# Autodesk Inventor assembly: ASSEMBLY_Main_XY_Axis
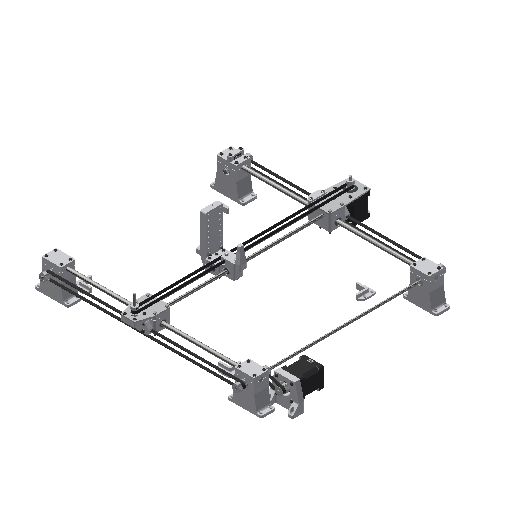
[picture p0: Inventor's stored thumbnail of the model, 512x512]
Saved by Autodesk Inventor 2025 (Build 290162010, 162A)
## iProperties
Created: 2018-06-17
Part Number: ASSEMBLY_Main_XY_Axis
Document SubType Name: Assembly
Designer: Andrzej
Author: Andrzej
## Documents named in this file (41)
- D:\_ANDRZEJ_LACZEWSKI\_OTHER\MLTDIS - SMD parts sorting machine experimental 2 axis platform\MCAD\1_REV1\ASSEMBLY_XY_AXIS_REVA\ASSEMBLY_Main_XY_Axis.iam
- D:\_ANDRZEJ_LACZEWSKI\_OTHER\MLTDIS - SMD parts sorting machine experimental 2 axis platform\MCAD\1_REV1\ASSEMBLY_XY_AXIS_REVA\CUT_STEEL_5x425mm_Linear_rod.ipt
- D:\_ANDRZEJ_LACZEWSKI\_OTHER\MLTDIS - SMD parts sorting machine experimental 2 axis platform\MCAD\1_REV1\ASSEMBLY_XY_AXIS_REVA\CUT_STEEL_6x395mm_Linear_rod.ipt
- D:\_ANDRZEJ_LACZEWSKI\_OTHER\MLTDIS - SMD parts sorting machine experimental 2 axis platform\MCAD\1_REV1\ASSEMBLY_XY_AXIS_REVA\ASSEMBLY_X_end.iam
- D:\_ANDRZEJ_LACZEWSKI\_OTHER\MLTDIS - SMD parts sorting machine experimental 2 axis platform\MCAD\1_REV1\ASSEMBLY_XY_AXIS_REVA\ASSEMBLY_X_axis_carriage.iam
- D:\_ANDRZEJ_LACZEWSKI\_OTHER\MLTDIS - SMD parts sorting machine experimental 2 axis platform\MCAD\1_REV1\ASSEMBLY_XY_AXIS_REVA\ASSEMBLY_Y_axis_motor.iam
- D:\_ANDRZEJ_LACZEWSKI\_OTHER\MLTDIS - SMD parts sorting machine experimental 2 axis platform\MCAD\1_REV1\__COTS_PARTS\COTS_GENERIC_GT2_16T_Pulley.ipt
- D:\_ANDRZEJ_LACZEWSKI\_OTHER\MLTDIS - SMD parts sorting machine experimental 2 axis platform\MCAD\1_REV1\ASSEMBLY_XY_AXIS_REVA\LC_ALU_3mm_X_axis_belt_idler_mount_plate.ipt
- D:\_ANDRZEJ_LACZEWSKI\_OTHER\MLTDIS - SMD parts sorting machine experimental 2 axis platform\MCAD\1_REV1\__COTS_PARTS\COTS_AST_695HZZ_Bearing.ipt
- D:\_ANDRZEJ_LACZEWSKI\_OTHER\MLTDIS - SMD parts sorting machine experimental 2 axis platform\MCAD\1_REV1\ASSEMBLY_XY_AXIS_REVA\3DP_PLA_X_axis_idler_bearing_block.ipt
- D:\_ANDRZEJ_LACZEWSKI\_OTHER\MLTDIS - SMD parts sorting machine experimental 2 axis platform\MCAD\1_REV1\ASSEMBLY_XY_AXIS_REVA\CUT_STEEL_5x37mm_Linear_rod.ipt
- D:\_ANDRZEJ_LACZEWSKI\_OTHER\MLTDIS - SMD parts sorting machine experimental 2 axis platform\MCAD\1_REV1\ASSEMBLY_XY_AXIS_REVA\3DP_PLA_X_axis_carriage_belt_mount.ipt
- D:\_ANDRZEJ_LACZEWSKI\_OTHER\MLTDIS - SMD parts sorting machine experimental 2 axis platform\MCAD\1_REV1\ASSEMBLY_XY_AXIS_REVA\3DP_PLA_X_axis_idler_shaft_locking_ring.ipt
- D:\_ANDRZEJ_LACZEWSKI\_OTHER\MLTDIS - SMD parts sorting machine experimental 2 axis platform\MCAD\1_REV1\ASSEMBLY_XY_AXIS_REVA\3DP_PLA_X_axis_idler_shaft_washer.ipt
- D:\_ANDRZEJ_LACZEWSKI\_OTHER\MLTDIS - SMD parts sorting machine experimental 2 axis platform\MCAD\1_REV1\__COTS_PARTS\COTS_OMRON_D2FS-FL_Endstop.ipt
- D:\_ANDRZEJ_LACZEWSKI\_OTHER\MLTDIS - SMD parts sorting machine experimental 2 axis platform\MCAD\1_REV1\__COTS_PARTS\COTS_GENERIC_NEMA_17_Stepper_motor.ipt
- D:\_ANDRZEJ_LACZEWSKI\_OTHER\MLTDIS - SMD parts sorting machine experimental 2 axis platform\MCAD\1_REV1\ASSEMBLY_XY_AXIS_REVA\ASSEMBLY_Y_axis_front_linear_shaft_mount.iam
- D:\_ANDRZEJ_LACZEWSKI\_OTHER\MLTDIS - SMD parts sorting machine experimental 2 axis platform\MCAD\1_REV1\ASSEMBLY_XY_AXIS_REVA\ASSEMBLY_Y_axis_linear_shaft_mount.iam
- D:\_ANDRZEJ_LACZEWSKI\_OTHER\MLTDIS - SMD parts sorting machine experimental 2 axis platform\MCAD\1_REV1\ASSEMBLY_XY_AXIS_REVA\CUT_STEEL_8x434mm_Linear_rod.ipt
- D:\_ANDRZEJ_LACZEWSKI\_OTHER\MLTDIS - SMD parts sorting machine experimental 2 axis platform\MCAD\1_REV1\__COTS_PARTS\COTS_GENERIC_GT2_Timing_belt_6mm_Y_axis.ipt
- D:\_ANDRZEJ_LACZEWSKI\_OTHER\MLTDIS - SMD parts sorting machine experimental 2 axis platform\MCAD\1_REV1\__COTS_PARTS\COTS_GENERIC_GT2_Timing_belt_6mm_X_axis.ipt
- D:\_ANDRZEJ_LACZEWSKI\_OTHER\MLTDIS - SMD parts sorting machine experimental 2 axis platform\MCAD\1_REV1\__COTS_PARTS\COTS_GENERIC_GT2_20T_Pulley.ipt
- D:\_ANDRZEJ_LACZEWSKI\_OTHER\MLTDIS - SMD parts sorting machine experimental 2 axis platform\MCAD\1_REV1\ASSEMBLY_XY_AXIS_REVA\3DP_PLA_Y_axis_drive_shaft_pulley_washer.ipt
- D:\_ANDRZEJ_LACZEWSKI\_OTHER\MLTDIS - SMD parts sorting machine experimental 2 axis platform\MCAD\1_REV1\__COTS_PARTS\COTS_GENERIC_GT2_Timing_belt_6mm_closed_loop_stepper.ipt
- D:\_ANDRZEJ_LACZEWSKI\_OTHER\MLTDIS - SMD parts sorting machine experimental 2 axis platform\MCAD\1_REV1\ASSEMBLY_XY_AXIS_REVA\LC_ALU_3mm_X_axis_stepper_mount_plate.ipt
- D:\_ANDRZEJ_LACZEWSKI\_OTHER\MLTDIS - SMD parts sorting machine experimental 2 axis platform\MCAD\1_REV1\__COTS_PARTS\COTS_GENERIC_Engraving_laser.ipt
- D:\_ANDRZEJ_LACZEWSKI\_OTHER\MLTDIS - SMD parts sorting machine experimental 2 axis platform\MCAD\1_REV1\ASSEMBLY_XY_AXIS_REVA\3DP_PLA_Y_axis_endstop_mount.ipt
- D:\_ANDRZEJ_LACZEWSKI\_OTHER\MLTDIS - SMD parts sorting machine experimental 2 axis platform\MCAD\1_REV1\ASSEMBLY_XY_AXIS_REVA\3DP_PLA_Y_axis_endstop_pushrod.ipt
- D:\_ANDRZEJ_LACZEWSKI\_OTHER\MLTDIS - SMD parts sorting machine experimental 2 axis platform\MCAD\1_REV1\ASSEMBLY_XY_AXIS_REVA\3DP_PLA_X_axis_endstop_mount.ipt
- D:\_ANDRZEJ_LACZEWSKI\_OTHER\MLTDIS - SMD parts sorting machine experimental 2 axis platform\MCAD\1_REV1\ASSEMBLY_XY_AXIS_REVA\3DP_PLA_Build_area_corner_barrier.ipt
- D:\_ANDRZEJ_LACZEWSKI\_OTHER\MLTDIS - SMD parts sorting machine experimental 2 axis platform\MCAD\1_REV1\ASSEMBLY_XY_AXIS_REVA\3DP_PLA_X_axis_carriage_laser_mount.ipt
- D:\_ANDRZEJ_LACZEWSKI\_OTHER\MLTDIS - SMD parts sorting machine experimental 2 axis platform\MCAD\1_REV1\ASSEMBLY_XY_AXIS_REVA\3DP_PLA_X_axis_carriage_laser_mount_clamp.ipt
- D:\_ANDRZEJ_LACZEWSKI\_OTHER\MLTDIS - SMD parts sorting machine experimental 2 axis platform\MCAD\1_REV1\__CONTENT_CENTER_PARTS\en-US\DIN 125-2  A\DIN 125-2 - A 3,2A.ipt
- D:\_ANDRZEJ_LACZEWSKI\_OTHER\MLTDIS - SMD parts sorting machine experimental 2 axis platform\MCAD\1_REV1\__CONTENT_CENTER_PARTS\en-US\ANSI B18.3.4M(2)\ANSI B18.3.4M - M3 x 0.5 x 40(1).ipt
- D:\_ANDRZEJ_LACZEWSKI\_OTHER\MLTDIS - SMD parts sorting machine experimental 2 axis platform\MCAD\1_REV1\__CONTENT_CENTER_PARTS\en-US\DIN 934\DIN 934 - M3 x 0,5.ipt
- D:\_ANDRZEJ_LACZEWSKI\_OTHER\MLTDIS - SMD parts sorting machine experimental 2 axis platform\MCAD\1_REV1\__CONTENT_CENTER_PARTS\en-US\ISO 7380-1\ISO 7380-1 - M3 x 10.ipt
- D:\_ANDRZEJ_LACZEWSKI\_OTHER\MLTDIS - SMD parts sorting machine experimental 2 axis platform\MCAD\1_REV1\__CONTENT_CENTER_PARTS\en-US\ISO 7380-1\ISO 7380-1 - M3 x 6.ipt
- D:\_ANDRZEJ_LACZEWSKI\_OTHER\MLTDIS - SMD parts sorting machine experimental 2 axis platform\MCAD\1_REV1\__CONTENT_CENTER_PARTS\en-US\ANSI B18.3.4M(2)\ANSI B18.3.4M - M3 x 0.5 x 35(1).ipt
- D:\_ANDRZEJ_LACZEWSKI\_OTHER\MLTDIS - SMD parts sorting machine experimental 2 axis platform\MCAD\1_REV1\__CONTENT_CENTER_PARTS\en-US\ISO 7380-1\ISO 7380-1 - M3 x 25.ipt
- D:\_ANDRZEJ_LACZEWSKI\_OTHER\MLTDIS - SMD parts sorting machine experimental 2 axis platform\MCAD\1_REV1\__CONTENT_CENTER_PARTS\en-US\ISO 7380-1\ISO 7380-1 - M3 x 30.ipt
- D:\_ANDRZEJ_LACZEWSKI\_OTHER\MLTDIS - SMD parts sorting machine experimental 2 axis platform\MCAD\1_REV1\__CONTENT_CENTER_PARTS\en-US\ISO 7380-1\ISO 7380-1 - M3 x 12.ipt
## Components (143 placed, 40 different names)
1. CUT_STEEL_6x395mm_Linear_rod:1 — Mate:41, Flush:5, Mate:45, Flush:36
2. CUT_STEEL_6x395mm_Linear_rod:2 — Mate:42, Flush:4, Mate:44, Mate:46
3. ASSEMBLY_X_end:2 [sub-assembly] — Mate:41, Mate:42, Flush:4, Flush:5, Mate:113, Mate:125, Flush:40, Flush:41, Mate:197, Mate:199
4. ASSEMBLY_X_end:3 [sub-assembly] — Mate:44, Mate:66, Flush:17, Flush:18, Mate:114, Flush:36, Mate:173, Mate:175, Mate:177, Mate:179, Mate:181, Mate:183, Mate:185, Mate:187, Mate:189, Mate:191
5. ASSEMBLY_X_axis_carriage:1 [sub-assembly] — Mate:45, Mate:46, Mate:79, Flush:23, Mate:141, Flush:49, Mate:142, Mate:149, Mate:150, Flush:64, Mate:151, Mate:214, Mate:216, Mate:226, Mate:227, Mate:228, Mate:229, Mate:230, Mate:231
6. ASSEMBLY_Y_axis_motor:1 [sub-assembly] — Flush:38, Mate:123, Flush:39
7. COTS_GENERIC_GT2_16T_Pulley:1 — Mate:117, Mate:128, Flush:43
8. LC_ALU_3mm_X_axis_belt_idler_mount_plate:1 — Mate:66, Flush:17, Flush:18, Mate:67, Flush:19, Mate:115, Mate:152, Mate:153, Mate:154, Mate:155, Mate:156, Mate:157, Mate:158, Mate:159, Mate:160, Mate:161, Mate:162, Mate:163, Mate:165, Mate:167, Mate:169, Mate:171, Mate:172, Mate:174, Mate:176, Mate:178, Mate:180, Mate:182, Mate:200, Mate:201, Mate:202, Mate:203, Mate:207
9. 3DP_PLA_X_axis_idler_bearing_block:1 — Mate:67, Flush:19, Mate:69, Mate:70, Mate:71, Mate:115, Mate:204, Mate:205, Mate:206, Mate:208
10. COTS_AST_695HZZ_Bearing:1 — Mate:69, Mate:70, Mate:72, Mate:83
11. COTS_AST_695HZZ_Bearing:2 — Mate:71, Mate:72, Mate:73, Mate:81
12. CUT_STEEL_5x37mm_Linear_rod:1 — Mate:73, Mate:74, Mate:80, Mate:82
13. COTS_GENERIC_GT2_16T_Pulley:2 — Mate:74, Mate:116, Mate:129, Mate:130, Flush:43
14. 3DP_PLA_X_axis_carriage_belt_mount:1 — Mate:79, Flush:23, Mate:149, Mate:209, Mate:210, Mate:211, Mate:212, Mate:213, Mate:215
15. 3DP_PLA_X_axis_idler_shaft_locking_ring:1 — Mate:80, Mate:81
16. 3DP_PLA_X_axis_idler_shaft_washer:1 — Mate:82, Mate:83, Mate:116
17. COTS_OMRON_D2FS-FL_Endstop:1 — Mate:141, Flush:49, Mate:145
18. COTS_OMRON_D2FS-FL_Endstop:2 — Mate:134, Mate:135, Flush:45
19. COTS_GENERIC_NEMA_17_Stepper_motor:1 — Mate:126, Flush:42, Mate:127, Mate:128
20. ASSEMBLY_Y_axis_front_linear_shaft_mount:1 [sub-assembly] — Flush:27, Flush:28, Flush:29, Mate:101, Flush:30, Mate:107, Mate:109, Flush:52, Flush:53, Flush:54, Flush:55
21. ASSEMBLY_Y_axis_front_linear_shaft_mount:2 [sub-assembly] — Flush:27, Mate:106, Flush:35, Mate:110, Mate:133, Flush:44, Mate:135, Flush:46
22. ASSEMBLY_Y_axis_linear_shaft_mount:1 [sub-assembly] — Flush:29, Mate:102, Flush:31, Mate:103, Flush:32, Mate:108, Mate:118, Flush:38
23. ASSEMBLY_Y_axis_linear_shaft_mount:2 [sub-assembly] — Flush:28, Mate:104, Mate:105, Flush:34, Mate:111, Mate:112
24. CUT_STEEL_8x434mm_Linear_rod:1 — Mate:105, Flush:34, Mate:106, Flush:35, Mate:113
25. CUT_STEEL_8x434mm_Linear_rod:2 — Mate:101, Flush:30, Mate:102, Flush:31, Mate:114
26. CUT_STEEL_5x425mm_Linear_rod:1 — Mate:103, Flush:32, Mate:104, Mate:119, Mate:120
27. COTS_GENERIC_GT2_Timing_belt_6mm_Y_axis:1 — Mate:107, Mate:108, Mate:109
28. COTS_GENERIC_GT2_Timing_belt_6mm_Y_axis:2 — Mate:110, Mate:111, Mate:112
29. COTS_GENERIC_GT2_Timing_belt_6mm_X_axis:1 — Mate:117, Mate:129, Mate:130
30. COTS_GENERIC_GT2_20T_Pulley:1 — Mate:120, Mate:121, Mate:122, Flush:39, Mate:124
31. 3DP_PLA_Y_axis_drive_shaft_pulley_washer:1 — Mate:118, Mate:119, Mate:121
32. COTS_GENERIC_GT2_Timing_belt_6mm_closed_loop_stepper:1 — Mate:122, Mate:123, Mate:124
33. LC_ALU_3mm_X_axis_stepper_mount_plate:1 — Mate:125, Flush:40, Flush:41, Mate:126, Flush:42, Mate:127, Mate:138, Mate:139, Mate:140, Mate:164, Mate:166, Mate:168, Mate:170, Mate:184, Mate:186, Mate:188, Mate:190, Insert:29, Insert:30, Insert:31, Insert:32
34. COTS_GENERIC_Engraving_laser:1 — Mate:147
35. 3DP_PLA_Y_axis_endstop_mount:1 — Mate:133, Flush:44, Mate:134, Flush:45, Flush:46, Insert:59, Insert:60
36. 3DP_PLA_Y_axis_endstop_pushrod:1 — Mate:138, Mate:139, Mate:140, Mate:192, Mate:193, Mate:194, Mate:195, Mate:196, Mate:198
37. 3DP_PLA_X_axis_endstop_mount:1 — Mate:142, Mate:145, Mate:226, Mate:227, Insert:55, Insert:56
38. 3DP_PLA_Build_area_corner_barrier:1 — Flush:52, Mate:143, Flush:56, Mate:144, Flush:59
39. 3DP_PLA_Build_area_corner_barrier:2 — Flush:53, Mate:143, Flush:56, Flush:58
40. 3DP_PLA_Build_area_corner_barrier:3 — Flush:54, Mate:144, Flush:57, Flush:59
41. 3DP_PLA_Build_area_corner_barrier:4 — Flush:55, Flush:57, Flush:58
42. 3DP_PLA_X_axis_carriage_laser_mount:1 — Mate:147, Mate:148, Flush:63, Mate:150, Flush:64, Mate:151, Insert:41, Insert:42, Insert:43, Insert:44, Mate:217, Mate:223, Mate:225
43. 3DP_PLA_X_axis_carriage_laser_mount_clamp:1 — Mate:148, Flush:63, Mate:217, Mate:218, Mate:219, Mate:220, Mate:221, Mate:222, Mate:224
44. DIN 125-2 A A 3,2:1 — Mate:152, Mate:153, Insert:1
45. Forged Hexagon Socket Button Head Cap Screw - Metric M3 x 0.5 x 40:1 — Insert:1
46. DIN 125-2 A A 3,2:2 — Mate:172, Mate:173, Insert:11
47. DIN 934 - replaced by DIN EN 24032/28673/28674 M3:1 — Insert:11
48. DIN 125-2 A A 3,2:3 — Mate:154, Mate:155, Insert:2
49. DIN 125-2 A A 3,2:4 — Mate:156, Mate:157, Insert:3
50. DIN 125-2 A A 3,2:5 — Mate:158, Mate:159, Insert:4
51. DIN 125-2 A A 3,2:6 — Mate:160, Mate:161, Insert:5
52. DIN 125-2 A A 3,2:7 — Mate:162, Mate:163, Insert:6
53. DIN 125-2 A A 3,2:8 — Mate:164, Mate:165, Insert:7
54. DIN 125-2 A A 3,2:9 — Mate:166, Mate:167, Insert:8
55. DIN 125-2 A A 3,2:10 — Mate:168, Mate:169, Insert:9
56. DIN 125-2 A A 3,2:11 — Mate:170, Mate:171, Insert:10
57. Forged Hexagon Socket Button Head Cap Screw - Metric M3 x 0.5 x 40:2 — Insert:2
58. Forged Hexagon Socket Button Head Cap Screw - Metric M3 x 0.5 x 40:3 — Insert:3
59. Forged Hexagon Socket Button Head Cap Screw - Metric M3 x 0.5 x 40:4 — Insert:4
60. Forged Hexagon Socket Button Head Cap Screw - Metric M3 x 0.5 x 40:5 — Insert:5
61. Forged Hexagon Socket Button Head Cap Screw - Metric M3 x 0.5 x 40:6 — Insert:6
62. Forged Hexagon Socket Button Head Cap Screw - Metric M3 x 0.5 x 40:7 — Insert:7
63. Forged Hexagon Socket Button Head Cap Screw - Metric M3 x 0.5 x 40:8 — Insert:8
64. Forged Hexagon Socket Button Head Cap Screw - Metric M3 x 0.5 x 40:9 — Insert:9
65. Forged Hexagon Socket Button Head Cap Screw - Metric M3 x 0.5 x 40:10 — Insert:10
66. DIN 125-2 A A 3,2:12 — Mate:174, Mate:175, Insert:12
67. DIN 125-2 A A 3,2:13 — Mate:176, Mate:177, Insert:13
68. DIN 125-2 A A 3,2:14 — Mate:178, Mate:179, Insert:14
69. DIN 125-2 A A 3,2:15 — Mate:180, Mate:181, Insert:15
70. DIN 125-2 A A 3,2:16 — Mate:182, Mate:183, Insert:16
71. DIN 125-2 A A 3,2:17 — Mate:184, Mate:185, Insert:17
72. DIN 125-2 A A 3,2:18 — Mate:186, Mate:187, Insert:18
73. DIN 125-2 A A 3,2:19 — Mate:188, Mate:189, Insert:19
74. DIN 125-2 A A 3,2:20 — Mate:190, Mate:191, Insert:20
75. DIN 934 - replaced by DIN EN 24032/28673/28674 M3:2 — Insert:12
76. DIN 934 - replaced by DIN EN 24032/28673/28674 M3:3 — Insert:13
77. DIN 934 - replaced by DIN EN 24032/28673/28674 M3:4 — Insert:14
78. DIN 934 - replaced by DIN EN 24032/28673/28674 M3:5 — Insert:15
79. DIN 934 - replaced by DIN EN 24032/28673/28674 M3:6 — Insert:16
80. DIN 934 - replaced by DIN EN 24032/28673/28674 M3:7 — Insert:17
81. DIN 934 - replaced by DIN EN 24032/28673/28674 M3:8 — Insert:18
82. DIN 934 - replaced by DIN EN 24032/28673/28674 M3:9 — Insert:19
83. DIN 934 - replaced by DIN EN 24032/28673/28674 M3:10 — Insert:20
84. DIN 125-2 A A 3,2:21 — Mate:192, Mate:193, Insert:21
85. Forged Hexagon Socket Button Head Cap Screw - Metric M3 x 0.5 x 40:11 — Insert:21
86. DIN 125-2 A A 3,2:22 — Mate:196, Mate:197, Insert:23
87. DIN 934 - replaced by DIN EN 24032/28673/28674 M3:11 — Insert:23
88. DIN 125-2 A A 3,2:23 — Mate:194, Mate:195, Insert:22
89. Forged Hexagon Socket Button Head Cap Screw - Metric M3 x 0.5 x 40:12 — Insert:22
90. DIN 125-2 A A 3,2:24 — Mate:198, Mate:199, Insert:24
91. DIN 934 - replaced by DIN EN 24032/28673/28674 M3:12 — Insert:24
92. DIN 125-2 A A 3,2:25 — Mate:203, Mate:206, Insert:25
93. DIN 125-2 A A 3,2:26 — Mate:202, Mate:207, Mate:208, Insert:28
94. DIN 125-2 A A 3,2:27 — Mate:201, Mate:205, Insert:27
95. DIN 125-2 A A 3,2:28 — Mate:200, Mate:204, Insert:26
96. ISO 7380-1 M3 x 10:1 — Insert:25
97. ISO 7380-1 M3 x 10:2 — Insert:26
98. ISO 7380-1 M3 x 10:3 — Insert:27
99. ISO 7380-1 M3 x 10:4 — Insert:28
100. DIN 125-2 A A 3,2:29 — Insert:29, Insert:33
101. DIN 125-2 A A 3,2:30 — Insert:30, Insert:34
102. DIN 125-2 A A 3,2:31 — Insert:31, Insert:36
103. DIN 125-2 A A 3,2:32 — Insert:32, Insert:35
104. ISO 7380-1 M3 x 6:1 — Insert:33
105. ISO 7380-1 M3 x 6:2 — Insert:34
106. ISO 7380-1 M3 x 6:3 — Insert:35
107. ISO 7380-1 M3 x 6:4 — Insert:36
108. DIN 125-2 A A 3,2:33 — Mate:209, Mate:210, Insert:37
109. Forged Hexagon Socket Button Head Cap Screw - Metric M3 x 0.5 x 35:1 — Insert:37
110. DIN 125-2 A A 3,2:34 — Mate:213, Mate:214, Insert:39
111. DIN 934 - replaced by DIN EN 24032/28673/28674 M3:13 — Insert:39
112. DIN 125-2 A A 3,2:35 — Mate:211, Mate:212, Insert:38
113. Forged Hexagon Socket Button Head Cap Screw - Metric M3 x 0.5 x 35:2 — Insert:38
114. DIN 125-2 A A 3,2:36 — Mate:215, Mate:216, Insert:40
115. DIN 934 - replaced by DIN EN 24032/28673/28674 M3:14 — Insert:40
116. DIN 125-2 A A 3,2:37 — Insert:41, Insert:48
117. DIN 125-2 A A 3,2:38 — Insert:42, Insert:46
118. DIN 125-2 A A 3,2:39 — Insert:43, Insert:47
119. DIN 125-2 A A 3,2:40 — Insert:44, Insert:45
120. ISO 7380-1 M3 x 10:5 — Insert:45
121. ISO 7380-1 M3 x 10:6 — Insert:46
122. ISO 7380-1 M3 x 10:7 — Insert:47
123. ISO 7380-1 M3 x 10:8 — Insert:48
124. DIN 125-2 A A 3,2:41 — Mate:218, Mate:219, Insert:49
125. ISO 7380-1 M3 x 25:1 — Insert:49
126. DIN 125-2 A A 3,2:42 — Mate:222, Mate:223, Insert:51
127. DIN 934 - replaced by DIN EN 24032/28673/28674 M3:15 — Insert:51
128. DIN 125-2 A A 3,2:43 — Mate:220, Mate:221, Insert:50
129. ISO 7380-1 M3 x 25:2 — Insert:50
130. DIN 125-2 A A 3,2:44 — Mate:224, Mate:225, Insert:52
131. DIN 934 - replaced by DIN EN 24032/28673/28674 M3:16 — Insert:52
132. DIN 125-2 A A 3,2:45 — Mate:228, Mate:229, Insert:53
133. ISO 7380-1 M3 x 30:1 — Insert:53
134. DIN 125-2 A A 3,2:46 — Mate:230, Mate:231, Insert:54
135. ISO 7380-1 M3 x 30:2 — Insert:54
136. DIN 125-2 A A 3,2:47 — Insert:55, Insert:57
137. DIN 125-2 A A 3,2:48 — Insert:56, Insert:58
138. DIN 934 - replaced by DIN EN 24032/28673/28674 M3:17 — Insert:57
139. DIN 934 - replaced by DIN EN 24032/28673/28674 M3:18 — Insert:58
140. DIN 125-2 A A 3,2:49 — Insert:59, Insert:61
141. DIN 125-2 A A 3,2:50 — Insert:60, Insert:62
142. ISO 7380-1 M3 x 12:1 — Insert:61
143. ISO 7380-1 M3 x 12:2 — Insert:62
## Relationships (241: Mate 144, Insert 62, Flush 35)
- Mate:41: CUT_STEEL_6x395mm_Linear_rod:1 ↔ ASSEMBLY_X_end:2
- Mate:42: CUT_STEEL_6x395mm_Linear_rod:2 ↔ ASSEMBLY_X_end:2
- Flush:4: CUT_STEEL_6x395mm_Linear_rod:2 ↔ ASSEMBLY_X_end:2
- Flush:5: CUT_STEEL_6x395mm_Linear_rod:1 ↔ ASSEMBLY_X_end:2
- Mate:44: CUT_STEEL_6x395mm_Linear_rod:2 ↔ ASSEMBLY_X_end:3
- Mate:45: CUT_STEEL_6x395mm_Linear_rod:1 ↔ ASSEMBLY_X_axis_carriage:1
- Mate:46: CUT_STEEL_6x395mm_Linear_rod:2 ↔ ASSEMBLY_X_axis_carriage:1
- Mate:66: ASSEMBLY_X_end:3 ↔ LC_ALU_3mm_X_axis_belt_idler_mount_plate:1
- Flush:17: ASSEMBLY_X_end:3 ↔ LC_ALU_3mm_X_axis_belt_idler_mount_plate:1
- Flush:18: ASSEMBLY_X_end:3 ↔ LC_ALU_3mm_X_axis_belt_idler_mount_plate:1
- Mate:67: LC_ALU_3mm_X_axis_belt_idler_mount_plate:1 ↔ 3DP_PLA_X_axis_idler_bearing_block:1
- Flush:19: LC_ALU_3mm_X_axis_belt_idler_mount_plate:1 ↔ 3DP_PLA_X_axis_idler_bearing_block:1
- Mate:69: 3DP_PLA_X_axis_idler_bearing_block:1 ↔ COTS_AST_695HZZ_Bearing:1
- Mate:70: 3DP_PLA_X_axis_idler_bearing_block:1 ↔ COTS_AST_695HZZ_Bearing:1
- Mate:71: 3DP_PLA_X_axis_idler_bearing_block:1 ↔ COTS_AST_695HZZ_Bearing:2
- Mate:72: COTS_AST_695HZZ_Bearing:1 ↔ COTS_AST_695HZZ_Bearing:2
- Mate:73: COTS_AST_695HZZ_Bearing:2 ↔ CUT_STEEL_5x37mm_Linear_rod:1
- Mate:74: CUT_STEEL_5x37mm_Linear_rod:1 ↔ COTS_GENERIC_GT2_16T_Pulley:2
- Mate:79: ASSEMBLY_X_axis_carriage:1 ↔ 3DP_PLA_X_axis_carriage_belt_mount:1
- Flush:23: ASSEMBLY_X_axis_carriage:1 ↔ 3DP_PLA_X_axis_carriage_belt_mount:1
- Mate:80: CUT_STEEL_5x37mm_Linear_rod:1 ↔ 3DP_PLA_X_axis_idler_shaft_locking_ring:1
- Mate:81: COTS_AST_695HZZ_Bearing:2 ↔ 3DP_PLA_X_axis_idler_shaft_locking_ring:1
- Mate:82: CUT_STEEL_5x37mm_Linear_rod:1 ↔ 3DP_PLA_X_axis_idler_shaft_washer:1
- Mate:83: COTS_AST_695HZZ_Bearing:1 ↔ 3DP_PLA_X_axis_idler_shaft_washer:1
- Flush:27: ASSEMBLY_Y_axis_front_linear_shaft_mount:1 ↔ ASSEMBLY_Y_axis_front_linear_shaft_mount:2
- Flush:28: ASSEMBLY_Y_axis_front_linear_shaft_mount:1 ↔ ASSEMBLY_Y_axis_linear_shaft_mount:2
- Flush:29: ASSEMBLY_Y_axis_front_linear_shaft_mount:1 ↔ ASSEMBLY_Y_axis_linear_shaft_mount:1
- Mate:101: ASSEMBLY_Y_axis_front_linear_shaft_mount:1 ↔ CUT_STEEL_8x434mm_Linear_rod:2
- Flush:30: ASSEMBLY_Y_axis_front_linear_shaft_mount:1 ↔ CUT_STEEL_8x434mm_Linear_rod:2
- Mate:102: ASSEMBLY_Y_axis_linear_shaft_mount:1 ↔ CUT_STEEL_8x434mm_Linear_rod:2
- Flush:31: ASSEMBLY_Y_axis_linear_shaft_mount:1 ↔ CUT_STEEL_8x434mm_Linear_rod:2
- Mate:103: ASSEMBLY_Y_axis_linear_shaft_mount:1 ↔ CUT_STEEL_5x425mm_Linear_rod:1
- Flush:32: ASSEMBLY_Y_axis_linear_shaft_mount:1 ↔ CUT_STEEL_5x425mm_Linear_rod:1
- Mate:104: ASSEMBLY_Y_axis_linear_shaft_mount:2 ↔ CUT_STEEL_5x425mm_Linear_rod:1
- Mate:105: ASSEMBLY_Y_axis_linear_shaft_mount:2 ↔ CUT_STEEL_8x434mm_Linear_rod:1
- Flush:34: ASSEMBLY_Y_axis_linear_shaft_mount:2 ↔ CUT_STEEL_8x434mm_Linear_rod:1
- Mate:106: ASSEMBLY_Y_axis_front_linear_shaft_mount:2 ↔ CUT_STEEL_8x434mm_Linear_rod:1
- Flush:35: ASSEMBLY_Y_axis_front_linear_shaft_mount:2 ↔ CUT_STEEL_8x434mm_Linear_rod:1
- Mate:107: ASSEMBLY_Y_axis_front_linear_shaft_mount:1 ↔ COTS_GENERIC_GT2_Timing_belt_6mm_Y_axis:1
- Mate:108: ASSEMBLY_Y_axis_linear_shaft_mount:1 ↔ COTS_GENERIC_GT2_Timing_belt_6mm_Y_axis:1
- Mate:109 (0.5 mm): ASSEMBLY_Y_axis_front_linear_shaft_mount:1 ↔ COTS_GENERIC_GT2_Timing_belt_6mm_Y_axis:1
- Mate:110: ASSEMBLY_Y_axis_front_linear_shaft_mount:2 ↔ COTS_GENERIC_GT2_Timing_belt_6mm_Y_axis:2
- Mate:111: ASSEMBLY_Y_axis_linear_shaft_mount:2 ↔ COTS_GENERIC_GT2_Timing_belt_6mm_Y_axis:2
- Mate:112 (0.5 mm): ASSEMBLY_Y_axis_linear_shaft_mount:2 ↔ COTS_GENERIC_GT2_Timing_belt_6mm_Y_axis:2
- Mate:113: ASSEMBLY_X_end:2 ↔ CUT_STEEL_8x434mm_Linear_rod:1
- Mate:114: ASSEMBLY_X_end:3 ↔ CUT_STEEL_8x434mm_Linear_rod:2
- Flush:36: CUT_STEEL_6x395mm_Linear_rod:1 ↔ ASSEMBLY_X_end:3
- Mate:115: LC_ALU_3mm_X_axis_belt_idler_mount_plate:1 ↔ 3DP_PLA_X_axis_idler_bearing_block:1
- Mate:116: COTS_GENERIC_GT2_16T_Pulley:2 ↔ 3DP_PLA_X_axis_idler_shaft_washer:1
- Mate:117: COTS_GENERIC_GT2_16T_Pulley:1 ↔ COTS_GENERIC_GT2_Timing_belt_6mm_X_axis:1
- Mate:118: ASSEMBLY_Y_axis_linear_shaft_mount:1 ↔ 3DP_PLA_Y_axis_drive_shaft_pulley_washer:1
- Mate:119: CUT_STEEL_5x425mm_Linear_rod:1 ↔ 3DP_PLA_Y_axis_drive_shaft_pulley_washer:1
- Mate:120: CUT_STEEL_5x425mm_Linear_rod:1 ↔ COTS_GENERIC_GT2_20T_Pulley:1
- Mate:121: COTS_GENERIC_GT2_20T_Pulley:1 ↔ 3DP_PLA_Y_axis_drive_shaft_pulley_washer:1
- Flush:38: ASSEMBLY_Y_axis_motor:1 ↔ ASSEMBLY_Y_axis_linear_shaft_mount:1
- Mate:122: COTS_GENERIC_GT2_20T_Pulley:1 ↔ COTS_GENERIC_GT2_Timing_belt_6mm_closed_loop_stepper:1
- Mate:123: ASSEMBLY_Y_axis_motor:1 ↔ COTS_GENERIC_GT2_Timing_belt_6mm_closed_loop_stepper:1
- Flush:39: ASSEMBLY_Y_axis_motor:1 ↔ COTS_GENERIC_GT2_20T_Pulley:1
- Mate:124 (0.75 mm): COTS_GENERIC_GT2_20T_Pulley:1 ↔ COTS_GENERIC_GT2_Timing_belt_6mm_closed_loop_stepper:1
- Mate:125: ASSEMBLY_X_end:2 ↔ LC_ALU_3mm_X_axis_stepper_mount_plate:1
- Flush:40: ASSEMBLY_X_end:2 ↔ LC_ALU_3mm_X_axis_stepper_mount_plate:1
- Flush:41: ASSEMBLY_X_end:2 ↔ LC_ALU_3mm_X_axis_stepper_mount_plate:1
- Mate:126: COTS_GENERIC_NEMA_17_Stepper_motor:1 ↔ LC_ALU_3mm_X_axis_stepper_mount_plate:1
- Flush:42: COTS_GENERIC_NEMA_17_Stepper_motor:1 ↔ LC_ALU_3mm_X_axis_stepper_mount_plate:1
- Mate:127: COTS_GENERIC_NEMA_17_Stepper_motor:1 ↔ LC_ALU_3mm_X_axis_stepper_mount_plate:1
- Mate:128: COTS_GENERIC_GT2_16T_Pulley:1 ↔ COTS_GENERIC_NEMA_17_Stepper_motor:1
- Mate:129: COTS_GENERIC_GT2_16T_Pulley:2 ↔ COTS_GENERIC_GT2_Timing_belt_6mm_X_axis:1
- Mate:130 (0.5 mm): COTS_GENERIC_GT2_16T_Pulley:2 ↔ COTS_GENERIC_GT2_Timing_belt_6mm_X_axis:1
- Flush:43: COTS_GENERIC_GT2_16T_Pulley:1 ↔ COTS_GENERIC_GT2_16T_Pulley:2
- Mate:133: ASSEMBLY_Y_axis_front_linear_shaft_mount:2 ↔ 3DP_PLA_Y_axis_endstop_mount:1
- Flush:44: ASSEMBLY_Y_axis_front_linear_shaft_mount:2 ↔ 3DP_PLA_Y_axis_endstop_mount:1
- Mate:134: COTS_OMRON_D2FS-FL_Endstop:2 ↔ 3DP_PLA_Y_axis_endstop_mount:1
- Mate:135: COTS_OMRON_D2FS-FL_Endstop:2 ↔ ASSEMBLY_Y_axis_front_linear_shaft_mount:2
- Flush:45: COTS_OMRON_D2FS-FL_Endstop:2 ↔ 3DP_PLA_Y_axis_endstop_mount:1
- Flush:46 (-12 mm): ASSEMBLY_Y_axis_front_linear_shaft_mount:2 ↔ 3DP_PLA_Y_axis_endstop_mount:1
- Mate:138: LC_ALU_3mm_X_axis_stepper_mount_plate:1 ↔ 3DP_PLA_Y_axis_endstop_pushrod:1
- Mate:139: LC_ALU_3mm_X_axis_stepper_mount_plate:1 ↔ 3DP_PLA_Y_axis_endstop_pushrod:1
- Mate:140: LC_ALU_3mm_X_axis_stepper_mount_plate:1 ↔ 3DP_PLA_Y_axis_endstop_pushrod:1
- Mate:141: ASSEMBLY_X_axis_carriage:1 ↔ COTS_OMRON_D2FS-FL_Endstop:1
- Flush:49: ASSEMBLY_X_axis_carriage:1 ↔ COTS_OMRON_D2FS-FL_Endstop:1
- Mate:142: ASSEMBLY_X_axis_carriage:1 ↔ 3DP_PLA_X_axis_endstop_mount:1
- Flush:52: ASSEMBLY_Y_axis_front_linear_shaft_mount:1 ↔ 3DP_PLA_Build_area_corner_barrier:1
- Flush:53: ASSEMBLY_Y_axis_front_linear_shaft_mount:1 ↔ 3DP_PLA_Build_area_corner_barrier:2
- Flush:54: ASSEMBLY_Y_axis_front_linear_shaft_mount:1 ↔ 3DP_PLA_Build_area_corner_barrier:3
- Flush:55: ASSEMBLY_Y_axis_front_linear_shaft_mount:1 ↔ 3DP_PLA_Build_area_corner_barrier:4
- Mate:143 (277 mm): 3DP_PLA_Build_area_corner_barrier:1 ↔ 3DP_PLA_Build_area_corner_barrier:2
- Flush:56: 3DP_PLA_Build_area_corner_barrier:1 ↔ 3DP_PLA_Build_area_corner_barrier:2
- Mate:144 (302 mm): 3DP_PLA_Build_area_corner_barrier:1 ↔ 3DP_PLA_Build_area_corner_barrier:3
- Flush:57: 3DP_PLA_Build_area_corner_barrier:3 ↔ 3DP_PLA_Build_area_corner_barrier:4
- Flush:58: 3DP_PLA_Build_area_corner_barrier:2 ↔ 3DP_PLA_Build_area_corner_barrier:4
- Flush:59: 3DP_PLA_Build_area_corner_barrier:1 ↔ 3DP_PLA_Build_area_corner_barrier:3
- Mate:145: COTS_OMRON_D2FS-FL_Endstop:1 ↔ 3DP_PLA_X_axis_endstop_mount:1
- Mate:147: COTS_GENERIC_Engraving_laser:1 ↔ 3DP_PLA_X_axis_carriage_laser_mount:1
- Mate:148 (0.3 mm): 3DP_PLA_X_axis_carriage_laser_mount:1 ↔ 3DP_PLA_X_axis_carriage_laser_mount_clamp:1
- Flush:63: 3DP_PLA_X_axis_carriage_laser_mount:1 ↔ 3DP_PLA_X_axis_carriage_laser_mount_clamp:1
- Mate:149: ASSEMBLY_X_axis_carriage:1 ↔ 3DP_PLA_X_axis_carriage_belt_mount:1
- Mate:150: ASSEMBLY_X_axis_carriage:1 ↔ 3DP_PLA_X_axis_carriage_laser_mount:1
- Flush:64 (1 mm): ASSEMBLY_X_axis_carriage:1 ↔ 3DP_PLA_X_axis_carriage_laser_mount:1
- Mate:151: ASSEMBLY_X_axis_carriage:1 ↔ 3DP_PLA_X_axis_carriage_laser_mount:1
- Mate:152: LC_ALU_3mm_X_axis_belt_idler_mount_plate:1 ↔ DIN 125-2 A A 3,2:1
- Mate:153: LC_ALU_3mm_X_axis_belt_idler_mount_plate:1 ↔ DIN 125-2 A A 3,2:1
- Mate:154: LC_ALU_3mm_X_axis_belt_idler_mount_plate:1 ↔ DIN 125-2 A A 3,2:3
- Mate:155: LC_ALU_3mm_X_axis_belt_idler_mount_plate:1 ↔ DIN 125-2 A A 3,2:3
- Mate:156: LC_ALU_3mm_X_axis_belt_idler_mount_plate:1 ↔ DIN 125-2 A A 3,2:4
- Mate:157: LC_ALU_3mm_X_axis_belt_idler_mount_plate:1 ↔ DIN 125-2 A A 3,2:4
- Mate:158: LC_ALU_3mm_X_axis_belt_idler_mount_plate:1 ↔ DIN 125-2 A A 3,2:5
- Mate:159: LC_ALU_3mm_X_axis_belt_idler_mount_plate:1 ↔ DIN 125-2 A A 3,2:5
- Mate:160: LC_ALU_3mm_X_axis_belt_idler_mount_plate:1 ↔ DIN 125-2 A A 3,2:6
- Mate:161: LC_ALU_3mm_X_axis_belt_idler_mount_plate:1 ↔ DIN 125-2 A A 3,2:6
- Mate:162: LC_ALU_3mm_X_axis_belt_idler_mount_plate:1 ↔ DIN 125-2 A A 3,2:7
- Mate:163: LC_ALU_3mm_X_axis_belt_idler_mount_plate:1 ↔ DIN 125-2 A A 3,2:7
- Mate:164: LC_ALU_3mm_X_axis_stepper_mount_plate:1 ↔ DIN 125-2 A A 3,2:8
- Mate:165: LC_ALU_3mm_X_axis_belt_idler_mount_plate:1 ↔ DIN 125-2 A A 3,2:8
- Mate:166: LC_ALU_3mm_X_axis_stepper_mount_plate:1 ↔ DIN 125-2 A A 3,2:9
- Mate:167: LC_ALU_3mm_X_axis_belt_idler_mount_plate:1 ↔ DIN 125-2 A A 3,2:9
- Mate:168: LC_ALU_3mm_X_axis_stepper_mount_plate:1 ↔ DIN 125-2 A A 3,2:10
- Mate:169: LC_ALU_3mm_X_axis_belt_idler_mount_plate:1 ↔ DIN 125-2 A A 3,2:10
- Mate:170: LC_ALU_3mm_X_axis_stepper_mount_plate:1 ↔ DIN 125-2 A A 3,2:11
- Mate:171: LC_ALU_3mm_X_axis_belt_idler_mount_plate:1 ↔ DIN 125-2 A A 3,2:11
- Insert:1: DIN 125-2 A A 3,2:1 ↔ Forged Hexagon Socket Button Head Cap Screw - Metric M3 x 0.5 x 40:1
- Insert:2: DIN 125-2 A A 3,2:3 ↔ Forged Hexagon Socket Button Head Cap Screw - Metric M3 x 0.5 x 40:2
- Insert:3: DIN 125-2 A A 3,2:4 ↔ Forged Hexagon Socket Button Head Cap Screw - Metric M3 x 0.5 x 40:3
- Insert:4: DIN 125-2 A A 3,2:5 ↔ Forged Hexagon Socket Button Head Cap Screw - Metric M3 x 0.5 x 40:4
- Insert:5: DIN 125-2 A A 3,2:6 ↔ Forged Hexagon Socket Button Head Cap Screw - Metric M3 x 0.5 x 40:5
- Insert:6: DIN 125-2 A A 3,2:7 ↔ Forged Hexagon Socket Button Head Cap Screw - Metric M3 x 0.5 x 40:6
- Insert:7: DIN 125-2 A A 3,2:8 ↔ Forged Hexagon Socket Button Head Cap Screw - Metric M3 x 0.5 x 40:7
- Insert:8: DIN 125-2 A A 3,2:9 ↔ Forged Hexagon Socket Button Head Cap Screw - Metric M3 x 0.5 x 40:8
- Insert:9: DIN 125-2 A A 3,2:10 ↔ Forged Hexagon Socket Button Head Cap Screw - Metric M3 x 0.5 x 40:9
- Insert:10: DIN 125-2 A A 3,2:11 ↔ Forged Hexagon Socket Button Head Cap Screw - Metric M3 x 0.5 x 40:10
- Mate:172: LC_ALU_3mm_X_axis_belt_idler_mount_plate:1 ↔ DIN 125-2 A A 3,2:2
- Mate:173: ASSEMBLY_X_end:3 ↔ DIN 125-2 A A 3,2:2
- Mate:174: LC_ALU_3mm_X_axis_belt_idler_mount_plate:1 ↔ DIN 125-2 A A 3,2:12
- Mate:175: ASSEMBLY_X_end:3 ↔ DIN 125-2 A A 3,2:12
- Mate:176: LC_ALU_3mm_X_axis_belt_idler_mount_plate:1 ↔ DIN 125-2 A A 3,2:13
- Mate:177: ASSEMBLY_X_end:3 ↔ DIN 125-2 A A 3,2:13
- Mate:178: LC_ALU_3mm_X_axis_belt_idler_mount_plate:1 ↔ DIN 125-2 A A 3,2:14
- Mate:179: ASSEMBLY_X_end:3 ↔ DIN 125-2 A A 3,2:14
- Mate:180: LC_ALU_3mm_X_axis_belt_idler_mount_plate:1 ↔ DIN 125-2 A A 3,2:15
- Mate:181: ASSEMBLY_X_end:3 ↔ DIN 125-2 A A 3,2:15
- Mate:182: LC_ALU_3mm_X_axis_belt_idler_mount_plate:1 ↔ DIN 125-2 A A 3,2:16
- Mate:183: ASSEMBLY_X_end:3 ↔ DIN 125-2 A A 3,2:16
- Mate:184: LC_ALU_3mm_X_axis_stepper_mount_plate:1 ↔ DIN 125-2 A A 3,2:17
- Mate:185: ASSEMBLY_X_end:3 ↔ DIN 125-2 A A 3,2:17
- Mate:186: LC_ALU_3mm_X_axis_stepper_mount_plate:1 ↔ DIN 125-2 A A 3,2:18
- Mate:187: ASSEMBLY_X_end:3 ↔ DIN 125-2 A A 3,2:18
- Mate:188: LC_ALU_3mm_X_axis_stepper_mount_plate:1 ↔ DIN 125-2 A A 3,2:19
- Mate:189: ASSEMBLY_X_end:3 ↔ DIN 125-2 A A 3,2:19
- Mate:190: LC_ALU_3mm_X_axis_stepper_mount_plate:1 ↔ DIN 125-2 A A 3,2:20
- Mate:191: ASSEMBLY_X_end:3 ↔ DIN 125-2 A A 3,2:20
- Insert:11: DIN 125-2 A A 3,2:2 ↔ DIN 934 - replaced by DIN EN 24032/28673/28674 M3:1
- Insert:12: DIN 125-2 A A 3,2:12 ↔ DIN 934 - replaced by DIN EN 24032/28673/28674 M3:2
- Insert:13: DIN 125-2 A A 3,2:13 ↔ DIN 934 - replaced by DIN EN 24032/28673/28674 M3:3
- Insert:14: DIN 125-2 A A 3,2:14 ↔ DIN 934 - replaced by DIN EN 24032/28673/28674 M3:4
- Insert:15: DIN 125-2 A A 3,2:15 ↔ DIN 934 - replaced by DIN EN 24032/28673/28674 M3:5
- Insert:16: DIN 125-2 A A 3,2:16 ↔ DIN 934 - replaced by DIN EN 24032/28673/28674 M3:6
- Insert:17: DIN 125-2 A A 3,2:17 ↔ DIN 934 - replaced by DIN EN 24032/28673/28674 M3:7
- Insert:18: DIN 125-2 A A 3,2:18 ↔ DIN 934 - replaced by DIN EN 24032/28673/28674 M3:8
- Insert:19: DIN 125-2 A A 3,2:19 ↔ DIN 934 - replaced by DIN EN 24032/28673/28674 M3:9
- Insert:20: DIN 125-2 A A 3,2:20 ↔ DIN 934 - replaced by DIN EN 24032/28673/28674 M3:10
- Mate:192: 3DP_PLA_Y_axis_endstop_pushrod:1 ↔ DIN 125-2 A A 3,2:21
- Mate:193: 3DP_PLA_Y_axis_endstop_pushrod:1 ↔ DIN 125-2 A A 3,2:21
- Mate:194: 3DP_PLA_Y_axis_endstop_pushrod:1 ↔ DIN 125-2 A A 3,2:23
- Mate:195: 3DP_PLA_Y_axis_endstop_pushrod:1 ↔ DIN 125-2 A A 3,2:23
- Insert:21: DIN 125-2 A A 3,2:21 ↔ Forged Hexagon Socket Button Head Cap Screw - Metric M3 x 0.5 x 40:11
- Insert:22: DIN 125-2 A A 3,2:23 ↔ Forged Hexagon Socket Button Head Cap Screw - Metric M3 x 0.5 x 40:12
- Mate:196: 3DP_PLA_Y_axis_endstop_pushrod:1 ↔ DIN 125-2 A A 3,2:22
- Mate:197: ASSEMBLY_X_end:2 ↔ DIN 125-2 A A 3,2:22
- Mate:198: 3DP_PLA_Y_axis_endstop_pushrod:1 ↔ DIN 125-2 A A 3,2:24
- Mate:199: ASSEMBLY_X_end:2 ↔ DIN 125-2 A A 3,2:24
- Insert:23: DIN 125-2 A A 3,2:22 ↔ DIN 934 - replaced by DIN EN 24032/28673/28674 M3:11
- Insert:24: DIN 125-2 A A 3,2:24 ↔ DIN 934 - replaced by DIN EN 24032/28673/28674 M3:12
- Mate:200: LC_ALU_3mm_X_axis_belt_idler_mount_plate:1 ↔ DIN 125-2 A A 3,2:28
- Mate:201: LC_ALU_3mm_X_axis_belt_idler_mount_plate:1 ↔ DIN 125-2 A A 3,2:27
- Mate:202: LC_ALU_3mm_X_axis_belt_idler_mount_plate:1 ↔ DIN 125-2 A A 3,2:26
- Mate:203: LC_ALU_3mm_X_axis_belt_idler_mount_plate:1 ↔ DIN 125-2 A A 3,2:25
- Mate:204: 3DP_PLA_X_axis_idler_bearing_block:1 ↔ DIN 125-2 A A 3,2:28
- Mate:205: 3DP_PLA_X_axis_idler_bearing_block:1 ↔ DIN 125-2 A A 3,2:27
- Mate:206: 3DP_PLA_X_axis_idler_bearing_block:1 ↔ DIN 125-2 A A 3,2:25
- Mate:207: LC_ALU_3mm_X_axis_belt_idler_mount_plate:1 ↔ DIN 125-2 A A 3,2:26
- Mate:208: 3DP_PLA_X_axis_idler_bearing_block:1 ↔ DIN 125-2 A A 3,2:26
- Insert:25: DIN 125-2 A A 3,2:25 ↔ ISO 7380-1 M3 x 10:1
- Insert:26: DIN 125-2 A A 3,2:28 ↔ ISO 7380-1 M3 x 10:2
- Insert:27: DIN 125-2 A A 3,2:27 ↔ ISO 7380-1 M3 x 10:3
- Insert:28: DIN 125-2 A A 3,2:26 ↔ ISO 7380-1 M3 x 10:4
- Insert:29: LC_ALU_3mm_X_axis_stepper_mount_plate:1 ↔ DIN 125-2 A A 3,2:29
- Insert:30: LC_ALU_3mm_X_axis_stepper_mount_plate:1 ↔ DIN 125-2 A A 3,2:30
- Insert:31: LC_ALU_3mm_X_axis_stepper_mount_plate:1 ↔ DIN 125-2 A A 3,2:31
- Insert:32: LC_ALU_3mm_X_axis_stepper_mount_plate:1 ↔ DIN 125-2 A A 3,2:32
- Insert:33: DIN 125-2 A A 3,2:29 ↔ ISO 7380-1 M3 x 6:1
- Insert:34: DIN 125-2 A A 3,2:30 ↔ ISO 7380-1 M3 x 6:2
- Insert:35: DIN 125-2 A A 3,2:32 ↔ ISO 7380-1 M3 x 6:3
- Insert:36: DIN 125-2 A A 3,2:31 ↔ ISO 7380-1 M3 x 6:4
- Mate:209: 3DP_PLA_X_axis_carriage_belt_mount:1 ↔ DIN 125-2 A A 3,2:33
- Mate:210: 3DP_PLA_X_axis_carriage_belt_mount:1 ↔ DIN 125-2 A A 3,2:33
- Mate:211: 3DP_PLA_X_axis_carriage_belt_mount:1 ↔ DIN 125-2 A A 3,2:35
- Mate:212: 3DP_PLA_X_axis_carriage_belt_mount:1 ↔ DIN 125-2 A A 3,2:35
- Insert:37: DIN 125-2 A A 3,2:33 ↔ Forged Hexagon Socket Button Head Cap Screw - Metric M3 x 0.5 x 35:1
- Insert:38: DIN 125-2 A A 3,2:35 ↔ Forged Hexagon Socket Button Head Cap Screw - Metric M3 x 0.5 x 35:2
- Mate:213: 3DP_PLA_X_axis_carriage_belt_mount:1 ↔ DIN 125-2 A A 3,2:34
- Mate:214: ASSEMBLY_X_axis_carriage:1 ↔ DIN 125-2 A A 3,2:34
- Mate:215: 3DP_PLA_X_axis_carriage_belt_mount:1 ↔ DIN 125-2 A A 3,2:36
- Mate:216: ASSEMBLY_X_axis_carriage:1 ↔ DIN 125-2 A A 3,2:36
- Insert:39: DIN 125-2 A A 3,2:34 ↔ DIN 934 - replaced by DIN EN 24032/28673/28674 M3:13
- Insert:40: DIN 125-2 A A 3,2:36 ↔ DIN 934 - replaced by DIN EN 24032/28673/28674 M3:14
- Insert:41: 3DP_PLA_X_axis_carriage_laser_mount:1 ↔ DIN 125-2 A A 3,2:37
- Insert:42: 3DP_PLA_X_axis_carriage_laser_mount:1 ↔ DIN 125-2 A A 3,2:38
- Insert:43: 3DP_PLA_X_axis_carriage_laser_mount:1 ↔ DIN 125-2 A A 3,2:39
- Insert:44: 3DP_PLA_X_axis_carriage_laser_mount:1 ↔ DIN 125-2 A A 3,2:40
- Insert:45: DIN 125-2 A A 3,2:40 ↔ ISO 7380-1 M3 x 10:5
- Insert:46: DIN 125-2 A A 3,2:38 ↔ ISO 7380-1 M3 x 10:6
- Insert:47: DIN 125-2 A A 3,2:39 ↔ ISO 7380-1 M3 x 10:7
- Insert:48: DIN 125-2 A A 3,2:37 ↔ ISO 7380-1 M3 x 10:8
- Mate:217: 3DP_PLA_X_axis_carriage_laser_mount:1 ↔ 3DP_PLA_X_axis_carriage_laser_mount_clamp:1
- Mate:218: 3DP_PLA_X_axis_carriage_laser_mount_clamp:1 ↔ DIN 125-2 A A 3,2:41
- Mate:219: 3DP_PLA_X_axis_carriage_laser_mount_clamp:1 ↔ DIN 125-2 A A 3,2:41
- Mate:220: 3DP_PLA_X_axis_carriage_laser_mount_clamp:1 ↔ DIN 125-2 A A 3,2:43
- Mate:221: 3DP_PLA_X_axis_carriage_laser_mount_clamp:1 ↔ DIN 125-2 A A 3,2:43
- Insert:49: DIN 125-2 A A 3,2:41 ↔ ISO 7380-1 M3 x 25:1
- Insert:50: DIN 125-2 A A 3,2:43 ↔ ISO 7380-1 M3 x 25:2
- Mate:222: 3DP_PLA_X_axis_carriage_laser_mount_clamp:1 ↔ DIN 125-2 A A 3,2:42
- Mate:223: 3DP_PLA_X_axis_carriage_laser_mount:1 ↔ DIN 125-2 A A 3,2:42
- Mate:224: 3DP_PLA_X_axis_carriage_laser_mount_clamp:1 ↔ DIN 125-2 A A 3,2:44
- Mate:225: 3DP_PLA_X_axis_carriage_laser_mount:1 ↔ DIN 125-2 A A 3,2:44
- Insert:51: DIN 125-2 A A 3,2:42 ↔ DIN 934 - replaced by DIN EN 24032/28673/28674 M3:15
- Insert:52: DIN 125-2 A A 3,2:44 ↔ DIN 934 - replaced by DIN EN 24032/28673/28674 M3:16
- Mate:226: ASSEMBLY_X_axis_carriage:1 ↔ 3DP_PLA_X_axis_endstop_mount:1
- Mate:227: ASSEMBLY_X_axis_carriage:1 ↔ 3DP_PLA_X_axis_endstop_mount:1
- Mate:228: ASSEMBLY_X_axis_carriage:1 ↔ DIN 125-2 A A 3,2:45
- Mate:229: ASSEMBLY_X_axis_carriage:1 ↔ DIN 125-2 A A 3,2:45
- Mate:230: ASSEMBLY_X_axis_carriage:1 ↔ DIN 125-2 A A 3,2:46
- Mate:231: ASSEMBLY_X_axis_carriage:1 ↔ DIN 125-2 A A 3,2:46
- Insert:53: DIN 125-2 A A 3,2:45 ↔ ISO 7380-1 M3 x 30:1
- Insert:54: DIN 125-2 A A 3,2:46 ↔ ISO 7380-1 M3 x 30:2
- Insert:55: 3DP_PLA_X_axis_endstop_mount:1 ↔ DIN 125-2 A A 3,2:47
- Insert:56: 3DP_PLA_X_axis_endstop_mount:1 ↔ DIN 125-2 A A 3,2:48
- Insert:57: DIN 125-2 A A 3,2:47 ↔ DIN 934 - replaced by DIN EN 24032/28673/28674 M3:17
- Insert:58: DIN 125-2 A A 3,2:48 ↔ DIN 934 - replaced by DIN EN 24032/28673/28674 M3:18
- Insert:59: 3DP_PLA_Y_axis_endstop_mount:1 ↔ DIN 125-2 A A 3,2:49
- Insert:60: 3DP_PLA_Y_axis_endstop_mount:1 ↔ DIN 125-2 A A 3,2:50
- Insert:61: DIN 125-2 A A 3,2:49 ↔ ISO 7380-1 M3 x 12:1
- Insert:62: DIN 125-2 A A 3,2:50 ↔ ISO 7380-1 M3 x 12:2
